# Autodesk Inventor assembly: ZMotor
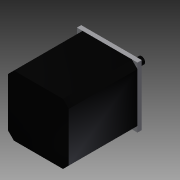
[picture p0: Inventor's stored thumbnail of the model, 180x180]
Saved by Autodesk Inventor 2015 (Build 190159000, 159)
## iProperties
Created: 2014-08-12
Part Number: ZMotor
Document SubType Name: Assembly
Designer: Jack
Author: Jack
## Documents named in this file (3)
- C:\Users\Jack\ownCloud\Projects\CoreXY\InventorModel\Old\ZAxis\ZMotor.old.iam
- C:\Users\Jack\ownCloud\Projects\CoreXY\InventorModel\Electronics\Motors\StepperMotorNema17.ipt
- C:\Users\Jack\ownCloud\Projects\CoreXY\InventorModel\Old\ZAxis\ZMotorMount.old.ipt
## Components (2 placed, 2 different names)
1. StepperMotorNema17:1 — Mate:1, Mate:2, Angle:1
2. ZMotorMount.old:1 — Mate:1, Mate:2, Angle:1
## Relationships (3: Mate 2, Angle 1)
- Mate:1: StepperMotorNema17:1 ↔ ZMotorMount.old:1
- Mate:2: StepperMotorNema17:1 ↔ ZMotorMount.old:1
- Angle:1 (0 deg): StepperMotorNema17:1 ↔ ZMotorMount.old:1
